# Autodesk Inventor assembly: Leg Assembly
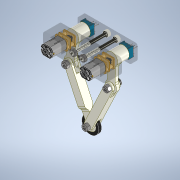
[picture p0: Inventor's stored thumbnail of the model, 180x180]
Saved by Autodesk Inventor 2022 (Build 260153000, 153)
## iProperties
Created: 2021-11-22
Part Number: Leg Assembly
Document SubType Name: Assembly
Designer: JK
Author: JK
## Documents named in this file (8)
- C:\Users\JK\Documents\Inventor\N20 Leg Actuator\CADfiles\Leg Assembly (small bearing).iam
- C:\Users\JK\Documents\Inventor\N20 Leg Actuator\CADfiles\Brushed DC Motor v8.iam
- C:\Users\JK\Documents\Inventor\N20 Leg Actuator\CADfiles\Base.ipt
- C:\Users\JK\Documents\Inventor\N20 Leg Actuator\CADfiles\Potenciometro10K.iam
- C:\Users\JK\Documents\Inventor\N20 Leg Actuator\CADfiles\PotHolder.ipt
- C:\Users\JK\Documents\Inventor\N20 Leg Actuator\CADfiles\m3x35.ipt
- C:\Users\JK\Documents\Inventor\N20 Leg Actuator\CADfiles\M3Nut.ipt
- C:\Users\JK\Documents\Inventor\N20 Leg Actuator\CADfiles\LegLinksAssembly.iam
## Components (11 placed, 7 different names)
1. Brushed DC Motor v8:1 [sub-assembly] — Coincidencia:2, Coincidencia:3, Ángulo:1
2. Brushed DC Motor v8:2 [sub-assembly] — Coincidencia:4, Ángulo:2, Coincidencia:5
3. Base:1 — Coincidencia:2, Coincidencia:3, Ángulo:1, Coincidencia:4, Ángulo:2, Coincidencia:5, Ángulo:4, Ángulo:5, Coincidencia:14, Coincidencia:36, Ángulo:7, Coincidencia:42
4. Potenciometro10K:1 [sub-assembly] — Nivelación:4, Ángulo:3, Ángulo:4, Nivelación:5
5. Potenciometro10K:2 [sub-assembly] — Nivelación:4, Ángulo:3
6. PotHolder:1 — Ángulo:5, Coincidencia:14, Nivelación:5, Coincidencia:36, Coincidencia:37, Coincidencia:38, Coincidencia:39
7. m3x35:1 — Coincidencia:37, Nivelación:17, Coincidencia:39, Coincidencia:40
8. m3x35:2 — Coincidencia:38, Nivelación:17, Coincidencia:41
9. M3Nut:1 — Coincidencia:40, Ángulo:6, Ángulo:7, Nivelación:18, Coincidencia:42
10. M3Nut:2 — Coincidencia:41, Ángulo:6, Nivelación:18
11. LegLinksAssembly:1 [sub-assembly]
## Relationships (29: Mate 18, Angle 7, Flush 4)
- Coincidencia:2 [Mate]: Brushed DC Motor v8:1 ↔ Base:1
- Coincidencia:3 [Mate]: Brushed DC Motor v8:1 ↔ Base:1
- Ángulo:1 [Angle] (0 deg): Brushed DC Motor v8:1 ↔ Base:1
- Coincidencia:4 [Mate]: Brushed DC Motor v8:2 ↔ Base:1
- Ángulo:2 [Angle] (0 deg): Brushed DC Motor v8:2 ↔ Base:1
- Coincidencia:5 [Mate]: Brushed DC Motor v8:2 ↔ Base:1
- [Mate]: Brushed DC Motor v8:2 ↔ LegLinksAssembly:1
- [Mate]: Brushed DC Motor v8:2 ↔ LegLinksAssembly:1
- [Mate]: Brushed DC Motor v8:1 ↔ LegLinksAssembly:1
- [Mate]: Potenciometro10K:1 ↔ LegLinksAssembly:1
- [Mate]: Brushed DC Motor v8:2 ↔ LegLinksAssembly:1
- Nivelación:4 [Flush]: Potenciometro10K:1 ↔ Potenciometro10K:2
- [Mate]: Potenciometro10K:2 ↔ LegLinksAssembly:1
- Ángulo:3 [Angle] (0 deg): Potenciometro10K:1 ↔ Potenciometro10K:2
- Ángulo:4 [Angle] (0 deg): Base:1 ↔ Potenciometro10K:1
- Ángulo:5 [Angle] (0 deg): Base:1 ↔ PotHolder:1
- Coincidencia:14 [Mate]: Base:1 ↔ PotHolder:1
- Nivelación:5 [Flush]: Potenciometro10K:1 ↔ PotHolder:1
- Coincidencia:36 [Mate]: Base:1 ↔ PotHolder:1
- Coincidencia:37 [Mate]: PotHolder:1 ↔ m3x35:1
- Coincidencia:38 [Mate]: PotHolder:1 ↔ m3x35:2
- Nivelación:17 [Flush]: m3x35:1 ↔ m3x35:2
- Coincidencia:39 [Mate]: PotHolder:1 ↔ m3x35:1
- Coincidencia:40 [Mate]: m3x35:1 ↔ M3Nut:1
- Coincidencia:41 [Mate]: m3x35:2 ↔ M3Nut:2
- Ángulo:6 [Angle] (0 deg): M3Nut:1 ↔ M3Nut:2
- Ángulo:7 [Angle] (0 deg): Base:1 ↔ M3Nut:1
- Nivelación:18 [Flush]: M3Nut:1 ↔ M3Nut:2
- Coincidencia:42 [Mate]: Base:1 ↔ M3Nut:1
